# Autodesk Inventor assembly: chassisstructure
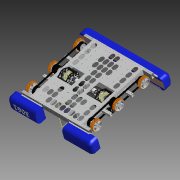
[picture p0: Inventor's stored thumbnail of the model, 180x180]
Saved by Autodesk Inventor 2014 SP1 (Build 180222100, 222)
## iProperties
Created: 2014-01-04
Part Number: chassisstructure
Document SubType Name: Assembly
Designer: Arpan
Mass: 5558.3 g
Surface Area: 28256.2 cm^2
Volume: 5506.27 cm^3
Density: 1.00945 g/cm^3
Author: Arpan
## Documents named in this file (25)
- C:\Users\Arpan\Documents\GitHub\2014buildCAD\chassisdrivetrain\chassis light\chassisstructure.iam
- C:\Users\Arpan\Documents\GitHub\2014buildCAD\chassisdrivetrain\chassis light\chassis side rail.ipt
- C:\Users\Arpan\Documents\GitHub\2014buildCAD\chassisdrivetrain\gearbot\3cimgearbox.iam
- C:\Users\Arpan\Documents\GitHub\2014buildCAD\chassisdrivetrain\chassis light\COTS items\center wheel assembly.iam
- C:\Users\Arpan\Documents\GitHub\2014buildCAD\chassisdrivetrain\chassis light\COTS items\.5 inch bearing pretend its hex.ipt
- C:\Users\Arpan\Documents\GitHub\2014buildCAD\chassisdrivetrain\chassis light\4.5 hex shaft.ipt
- C:\Users\Arpan\Documents\GitHub\2014buildCAD\chassisdrivetrain\chassis light\COTS items\front wheels.iam
- C:\Users\Arpan\Documents\GitHub\2014buildCAD\chassisdrivetrain\chassis light\COTS items\back wheels.iam
- C:\Users\Arpan\Documents\GitHub\2014buildCAD\chassisdrivetrain\chassis light\COTS items\DBK_42ToothPulley V2.iam
- C:\Users\Arpan\Documents\GitHub\2014buildCAD\chassisdrivetrain\chassis light\3d printed items\back wheel spacer.ipt
- C:\Users\Arpan\Documents\GitHub\2014buildCAD\chassisdrivetrain\chassis light\PVC pipe spacer.ipt
- C:\Users\Arpan\Documents\GitHub\2014buildCAD\chassisdrivetrain\chassis light\PVC pipe spacer center wheels.ipt
- C:\Users\Arpan\Documents\GitHub\2014buildCAD\chassisdrivetrain\chassis light\baseplate.ipt
- C:\Users\Arpan\Documents\GitHub\2014buildCAD\chassisdrivetrain\chassis light\battery mount.ipt
- C:\Users\Arpan\Documents\GitHub\2014buildCAD\chassisdrivetrain\chassis light\side bumper mount.ipt
- C:\Users\Arpan\Documents\GitHub\2014buildCAD\chassisdrivetrain\chassis light\COTS items\217-3547-STEP.ipt
- C:\Users\Arpan\Documents\GitHub\2014buildCAD\chassisdrivetrain\chassis light\front back rail vexpro.ipt
- C:\Users\Arpan\Documents\GitHub\2014buildCAD\chassisdrivetrain\chassis light\back rail vexpro.ipt
- C:\Users\Arpan\Documents\GitHub\2014buildCAD\chassisdrivetrain\chassis light\COTS items\HTD 5M-15 Belt 670mm.ipt
- C:\Users\Arpan\Documents\GitHub\2014buildCAD\chassisdrivetrain\chassis light\COTS items\HTD 5M-15 Belt 740mm.ipt
- C:\Users\Arpan\Documents\GitHub\2014buildCAD\chassisdrivetrain\chassis light\wheelhubthing.ipt
- C:\Users\Arpan\Documents\GitHub\2014buildCAD\chassisdrivetrain\chassis light\PVC pipe spacer front wheels.ipt
- C:\Users\Arpan\Documents\GitHub\2014buildCAD\Bumpers\Bumper Assembly2 (26x28 robot).iam
- C:\Users\Arpan\Documents\GitHub\2014buildCAD\Bumpers\Bumper Assembly3 (26x28 robot).iam
- C:\Users\Arpan\Documents\GitHub\2014buildCAD\Bumpers\Bumper Assembly4 (26x28 robot).iam
## Components (53 placed, 24 different names)
1. chassis side rail:1 — Mate:6, Mate:7, Mate:14, Mate:15, Mate:16, Mate:17, Mate:18, Mate:19, Mate:20, Mate:29, Mate:67, Mate:72, Flush:28, Mate:73, Flush:29, Mate:75, Flush:31, Flush:33, Mate:83, Flush:41, Flush:43, Flush:44, Mate:92, Mate:94, Mate:95, Mate:100, Mate:101
2. chassis side rail:2 — Mate:8, Mate:9, Mate:21, Mate:22, Mate:23, Mate:24, Mate:25, Mate:26, Mate:27, Mate:28, Angle:3, Flush:25, Mate:70, Mate:71, Flush:26, Flush:27, Flush:36, Mate:78, Flush:37, Mate:82, Flush:39, Mate:86, Flush:43, Mate:97, Mate:98, Mate:103, Mate:104
3. 3cimgearbox:1 [sub-assembly] — Mate:6, Mate:7, Angle:2, Flush:7, Mate:12, Mate:13, Mate:113
4. 3cimgearbox:2 [sub-assembly] — Mate:8, Mate:9, Angle:2, Flush:6, Mate:10, Mate:11, Angle:4, Mate:115
5. center wheel assembly:1 [sub-assembly] — Flush:6, Mate:10, Mate:11, Flush:17, Flush:18, Flush:22, Mate:114
6. center wheel assembly:2 [sub-assembly] — Flush:7, Mate:12, Mate:13, Flush:21, Flush:23, Mate:112
7. .5 inch bearing pretend its hex:1 — Mate:16, Mate:17
8. .5 inch bearing pretend its hex:2 — Mate:14, Mate:15, Mate:30
9. .5 inch bearing pretend its hex:3 — Mate:19, Mate:29
10. .5 inch bearing pretend its hex:4 — Mate:18, Mate:20, Mate:31
11. .5 inch bearing pretend its hex:5 — Mate:21, Mate:24, Mate:33
12. .5 inch bearing pretend its hex:6 — Mate:22, Mate:23
13. .5 inch bearing pretend its hex:7 — Mate:25, Mate:26, Mate:32
14. .5 inch bearing pretend its hex:8 — Mate:27, Mate:28
15. 4.5 hex shaft:1 — Mate:30, Flush:9, Flush:13, Mate:36, Mate:37, Mate:119
16. 4.5 hex shaft:2 — Mate:31, Flush:9, Flush:15, Mate:40, Mate:41, Mate:123
17. 4.5 hex shaft:3 — Mate:32, Flush:11, Mate:34, Mate:35, Angle:3, Flush:19, Mate:117
18. 4.5 hex shaft:4 — Flush:11, Mate:33, Mate:38, Mate:39, Flush:20, Mate:121
19. front wheels:1 [sub-assembly] — Mate:34, Mate:35, Flush:17, Flush:19, Mate:99, Mate:116
20. front wheels:2 [sub-assembly] — Flush:13, Mate:36, Mate:37, Flush:21, Mate:96, Mate:118
21. back wheels:1 [sub-assembly] — Flush:15, Mate:40, Mate:41, Mate:42, Mate:43, Mate:44, Mate:48, Mate:49, Mate:106, Mate:107
22. back wheels:2 [sub-assembly] — Mate:38, Mate:39, Mate:45, Mate:46, Flush:18, Flush:20, Mate:51, Mate:52, Mate:109, Mate:110
23. DBK_42ToothPulley V2:1 [sub-assembly] — Mate:42, Mate:43, Mate:44, Flush:23, Mate:47, Mate:102, Mate:108
24. DBK_42ToothPulley V2:2 [sub-assembly] — Mate:45, Mate:46, Flush:22, Mate:50, Mate:105, Mate:111
25. back wheel spacer:1 — Mate:47, Mate:48, Mate:49
26. back wheel spacer:2 — Mate:50, Mate:51, Mate:52
27. baseplate:1 — Flush:25, Mate:79, Mate:80, Mate:81, Flush:40, Mate:86, Mate:91, Flush:48
28. battery mount:1 — Mate:67, Mate:79, Mate:93
29. side bumper mount:1 — Mate:70, Flush:27, Flush:30, Mate:77, Flush:35, Mate:90
30. side bumper mount:2 — Mate:71, Flush:26, Flush:38, Flush:45, Mate:90, Flush:46
31. side bumper mount:3 — Mate:72, Flush:28, Flush:30, Flush:32
32. side bumper mount:4 — Mate:73, Flush:29, Mate:76, Flush:34, Flush:45
33. 217-3547-STEP:1 — Mate:75, Flush:31, Flush:32
34. 217-3547-STEP:2 — Mate:76, Flush:33, Flush:34
35. 217-3547-STEP:3 — Mate:77, Flush:35, Flush:36
36. 217-3547-STEP:4 — Mate:78, Flush:37, Flush:38
37. front back rail vexpro:1 — Mate:80, Mate:81, Mate:82, Flush:39, Mate:83, Flush:40, Flush:41, Flush:44, Flush:46, Flush:47, Mate:124, Flush:49
38. back rail vexpro:1 — Mate:91, Flush:47, Mate:92, Mate:93, Angle:4, Mate:125, Mate:126
39. HTD 5M-15 Belt 670mm:1 — Mate:100, Mate:101, Mate:102
40. HTD 5M-15 Belt 670mm:2 — Mate:103, Mate:104, Mate:105
41. HTD 5M-15 Belt 740mm:1 — Mate:94, Mate:95, Mate:96
42. HTD 5M-15 Belt 740mm:2 — Mate:97, Mate:98, Mate:99
43. wheelhubthing:1 — Mate:106, Mate:107, Mate:108, Mate:122
44. wheelhubthing:2 — Mate:109, Mate:110, Mate:111, Mate:120
45. PVC pipe spacer center wheels:1 — Mate:114, Mate:115
46. PVC pipe spacer center wheels:2 — Mate:112, Mate:113
47. PVC pipe spacer front wheels:1 — Mate:116, Mate:117
48. PVC pipe spacer front wheels:2 — Mate:118, Mate:119
49. PVC pipe spacer:1 — Mate:120, Mate:121
50. PVC pipe spacer:2 — Mate:122, Mate:123
51. Bumper Assembly2 (26x28 robot):1 [sub-assembly] — Mate:124, Flush:48, Flush:49, Flush:50, Flush:51, Flush:52, Flush:53
52. Bumper Assembly3 (26x28 robot):1 [sub-assembly] — Mate:126, Flush:50, Flush:53
53. Bumper Assembly4 (26x28 robot):1 [sub-assembly] — Mate:125, Flush:51, Flush:52
## Relationships (143: Mate 99, Flush 41, Angle 3)
- Mate:6: chassis side rail:1 ↔ 3cimgearbox:1
- Mate:7: chassis side rail:1 ↔ 3cimgearbox:1
- Mate:8: chassis side rail:2 ↔ 3cimgearbox:2
- Mate:9: chassis side rail:2 ↔ 3cimgearbox:2
- Angle:2 (0 deg): 3cimgearbox:1 ↔ 3cimgearbox:2
- Flush:6: 3cimgearbox:2 ↔ center wheel assembly:1
- Mate:10: 3cimgearbox:2 ↔ center wheel assembly:1
- Mate:11: 3cimgearbox:2 ↔ center wheel assembly:1
- Flush:7: 3cimgearbox:1 ↔ center wheel assembly:2
- Mate:12: 3cimgearbox:1 ↔ center wheel assembly:2
- Mate:13: 3cimgearbox:1 ↔ center wheel assembly:2
- Mate:14: chassis side rail:1 ↔ .5 inch bearing pretend its hex:2
- Mate:15: chassis side rail:1 ↔ .5 inch bearing pretend its hex:2
- Mate:16: chassis side rail:1 ↔ .5 inch bearing pretend its hex:1
- Mate:17: chassis side rail:1 ↔ .5 inch bearing pretend its hex:1
- Mate:18: chassis side rail:1 ↔ .5 inch bearing pretend its hex:4
- Mate:19: chassis side rail:1 ↔ .5 inch bearing pretend its hex:3
- Mate:20: chassis side rail:1 ↔ .5 inch bearing pretend its hex:4
- Mate:21: chassis side rail:2 ↔ .5 inch bearing pretend its hex:5
- Mate:22: chassis side rail:2 ↔ .5 inch bearing pretend its hex:6
- Mate:23: chassis side rail:2 ↔ .5 inch bearing pretend its hex:6
- Mate:24: chassis side rail:2 ↔ .5 inch bearing pretend its hex:5
- Mate:25: chassis side rail:2 ↔ .5 inch bearing pretend its hex:7
- Mate:26: chassis side rail:2 ↔ .5 inch bearing pretend its hex:7
- Mate:27: chassis side rail:2 ↔ .5 inch bearing pretend its hex:8
- Mate:28: chassis side rail:2 ↔ .5 inch bearing pretend its hex:8
- Mate:29: chassis side rail:1 ↔ .5 inch bearing pretend its hex:3
- Mate:30: .5 inch bearing pretend its hex:2 ↔ 4.5 hex shaft:1
- Mate:31: .5 inch bearing pretend its hex:4 ↔ 4.5 hex shaft:2
- Flush:9: 4.5 hex shaft:1 ↔ 4.5 hex shaft:2
- Mate:32: .5 inch bearing pretend its hex:7 ↔ 4.5 hex shaft:3
- Flush:11: 4.5 hex shaft:3 ↔ 4.5 hex shaft:4
- Mate:33: .5 inch bearing pretend its hex:5 ↔ 4.5 hex shaft:4
- Mate:34: 4.5 hex shaft:3 ↔ front wheels:1
- Mate:35: 4.5 hex shaft:3 ↔ front wheels:1
- Flush:13: 4.5 hex shaft:1 ↔ front wheels:2
- Mate:36: 4.5 hex shaft:1 ↔ front wheels:2
- Mate:37: 4.5 hex shaft:1 ↔ front wheels:2
- Mate:38: 4.5 hex shaft:4 ↔ back wheels:2
- Mate:39: 4.5 hex shaft:4 ↔ back wheels:2
- Flush:15: 4.5 hex shaft:2 ↔ back wheels:1
- Mate:40: 4.5 hex shaft:2 ↔ back wheels:1
- Mate:41: 4.5 hex shaft:2 ↔ back wheels:1
- Mate:42: back wheels:1 ↔ DBK_42ToothPulley V2:1
- Mate:43: back wheels:1 ↔ DBK_42ToothPulley V2:1
- Mate:44: back wheels:1 ↔ DBK_42ToothPulley V2:1
- Mate:45: back wheels:2 ↔ DBK_42ToothPulley V2:2
- Mate:46: back wheels:2 ↔ DBK_42ToothPulley V2:2
- Flush:17: center wheel assembly:1 ↔ front wheels:1
- Flush:18: center wheel assembly:1 ↔ back wheels:2
- Angle:3 (0 deg): chassis side rail:2 ↔ 4.5 hex shaft:3
- Flush:19: 4.5 hex shaft:3 ↔ front wheels:1
- Flush:20: 4.5 hex shaft:4 ↔ back wheels:2
- Flush:21: center wheel assembly:2 ↔ front wheels:2
- Flush:22: center wheel assembly:1 ↔ DBK_42ToothPulley V2:2
- Flush:23: center wheel assembly:2 ↔ DBK_42ToothPulley V2:1
- Mate:47: DBK_42ToothPulley V2:1 ↔ back wheel spacer:1
- Mate:48: back wheels:1 ↔ back wheel spacer:1
- Mate:49: back wheels:1 ↔ back wheel spacer:1
- Mate:50: DBK_42ToothPulley V2:2 ↔ back wheel spacer:2
- Mate:51: back wheels:2 ↔ back wheel spacer:2
- Mate:52: back wheels:2 ↔ back wheel spacer:2
- Flush:25: chassis side rail:2 ↔ baseplate:1
- Mate:67 (49.53 mm): chassis side rail:1 ↔ battery mount:1
- Mate:70: chassis side rail:2 ↔ side bumper mount:1
- Mate:71: chassis side rail:2 ↔ side bumper mount:2
- Flush:26: chassis side rail:2 ↔ side bumper mount:2
- Flush:27: chassis side rail:2 ↔ side bumper mount:1
- Mate:72: chassis side rail:1 ↔ side bumper mount:3
- Flush:28: chassis side rail:1 ↔ side bumper mount:3
- Mate:73: chassis side rail:1 ↔ side bumper mount:4
- Flush:29: chassis side rail:1 ↔ side bumper mount:4
- Flush:30: side bumper mount:1 ↔ side bumper mount:3
- Mate:75: chassis side rail:1 ↔ 217-3547-STEP:1
- Flush:31: chassis side rail:1 ↔ 217-3547-STEP:1
- Flush:32: side bumper mount:3 ↔ 217-3547-STEP:1
- Mate:76: side bumper mount:4 ↔ 217-3547-STEP:2
- Flush:33: chassis side rail:1 ↔ 217-3547-STEP:2
- Flush:34: side bumper mount:4 ↔ 217-3547-STEP:2
- Mate:77: side bumper mount:1 ↔ 217-3547-STEP:3
- Flush:35: side bumper mount:1 ↔ 217-3547-STEP:3
- Flush:36: chassis side rail:2 ↔ 217-3547-STEP:3
- Mate:78: chassis side rail:2 ↔ 217-3547-STEP:4
- Flush:37: chassis side rail:2 ↔ 217-3547-STEP:4
- Flush:38: side bumper mount:2 ↔ 217-3547-STEP:4
- Mate:79: baseplate:1 ↔ battery mount:1
- Mate:80: baseplate:1 ↔ front back rail vexpro:1
- Mate:81: baseplate:1 ↔ front back rail vexpro:1
- Mate:82: chassis side rail:2 ↔ front back rail vexpro:1
- Flush:39 (86.36 mm): chassis side rail:2 ↔ front back rail vexpro:1
- Mate:83: chassis side rail:1 ↔ front back rail vexpro:1
- Flush:40: baseplate:1 ↔ front back rail vexpro:1
- Flush:41: chassis side rail:1 ↔ front back rail vexpro:1
- Mate:86: chassis side rail:2 ↔ baseplate:1
- Flush:43: chassis side rail:1 ↔ chassis side rail:2
- Flush:44 (86.36 mm): chassis side rail:1 ↔ front back rail vexpro:1
- Flush:45: side bumper mount:2 ↔ side bumper mount:4
- Mate:90 (203.2 mm): side bumper mount:1 ↔ side bumper mount:2
- Flush:46 (-444.5 mm): side bumper mount:2 ↔ front back rail vexpro:1
- Mate:91: baseplate:1 ↔ back rail vexpro:1
- Flush:47: front back rail vexpro:1 ↔ back rail vexpro:1
- Mate:92: chassis side rail:1 ↔ back rail vexpro:1
- Mate:93: battery mount:1 ↔ back rail vexpro:1
- Mate:94: chassis side rail:1 ↔ HTD 5M-15 Belt 740mm:1
- Mate:95: chassis side rail:1 ↔ HTD 5M-15 Belt 740mm:1
- Mate:96 (0.7937 mm): front wheels:2 ↔ HTD 5M-15 Belt 740mm:1
- Mate:97: chassis side rail:2 ↔ HTD 5M-15 Belt 740mm:2
- Mate:98: chassis side rail:2 ↔ HTD 5M-15 Belt 740mm:2
- Mate:99 (0.7937 mm): front wheels:1 ↔ HTD 5M-15 Belt 740mm:2
- Mate:100: chassis side rail:1 ↔ HTD 5M-15 Belt 670mm:1
- Mate:101: chassis side rail:1 ↔ HTD 5M-15 Belt 670mm:1
- Mate:102 (0.7937 mm): DBK_42ToothPulley V2:1 ↔ HTD 5M-15 Belt 670mm:1
- Mate:103: chassis side rail:2 ↔ HTD 5M-15 Belt 670mm:2
- Mate:104: chassis side rail:2 ↔ HTD 5M-15 Belt 670mm:2
- Mate:105 (0.7937 mm): DBK_42ToothPulley V2:2 ↔ HTD 5M-15 Belt 670mm:2
- Angle:4 (0 deg): 3cimgearbox:2 ↔ back rail vexpro:1
- Mate:106: back wheels:1 ↔ wheelhubthing:1
- Mate:107: back wheels:1 ↔ wheelhubthing:1
- Mate:108: DBK_42ToothPulley V2:1 ↔ wheelhubthing:1
- Mate:109: back wheels:2 ↔ wheelhubthing:2
- Mate:110: back wheels:2 ↔ wheelhubthing:2
- Mate:111: DBK_42ToothPulley V2:2 ↔ wheelhubthing:2
- Mate:112: center wheel assembly:2 ↔ PVC pipe spacer center wheels:2
- Mate:113: 3cimgearbox:1 ↔ PVC pipe spacer center wheels:2
- Mate:114: center wheel assembly:1 ↔ PVC pipe spacer center wheels:1
- Mate:115: 3cimgearbox:2 ↔ PVC pipe spacer center wheels:1
- Mate:116: front wheels:1 ↔ PVC pipe spacer front wheels:1
- Mate:117: 4.5 hex shaft:3 ↔ PVC pipe spacer front wheels:1
- Mate:118: front wheels:2 ↔ PVC pipe spacer front wheels:2
- Mate:119: 4.5 hex shaft:1 ↔ PVC pipe spacer front wheels:2
- Mate:120: wheelhubthing:2 ↔ PVC pipe spacer:1
- Mate:121: 4.5 hex shaft:4 ↔ PVC pipe spacer:1
- Mate:122: wheelhubthing:1 ↔ PVC pipe spacer:2
- Mate:123: 4.5 hex shaft:2 ↔ PVC pipe spacer:2
- Mate:124: front back rail vexpro:1 ↔ Bumper Assembly2 (26x28 robot):1
- Flush:48 (25.4 mm): baseplate:1 ↔ Bumper Assembly2 (26x28 robot):1
- Flush:49 (-84.1375 mm): front back rail vexpro:1 ↔ Bumper Assembly2 (26x28 robot):1
- Mate:125: back rail vexpro:1 ↔ Bumper Assembly4 (26x28 robot):1
- Mate:126: back rail vexpro:1 ↔ Bumper Assembly3 (26x28 robot):1
- Flush:50: Bumper Assembly2 (26x28 robot):1 ↔ Bumper Assembly3 (26x28 robot):1
- Flush:51: Bumper Assembly2 (26x28 robot):1 ↔ Bumper Assembly4 (26x28 robot):1
- Flush:52: Bumper Assembly2 (26x28 robot):1 ↔ Bumper Assembly4 (26x28 robot):1
- Flush:53: Bumper Assembly2 (26x28 robot):1 ↔ Bumper Assembly3 (26x28 robot):1
